# Autodesk Inventor assembly: encoder
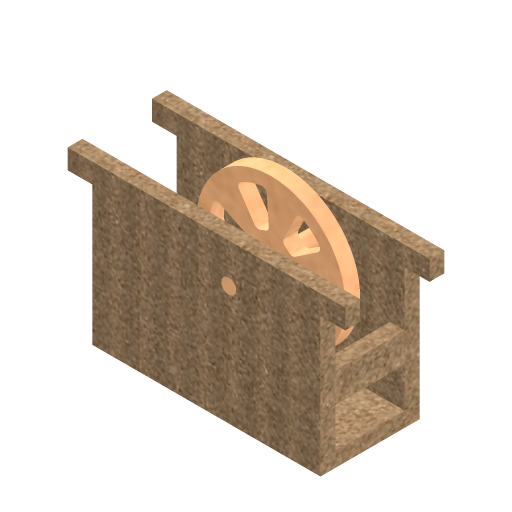
[picture p0: Inventor's stored thumbnail of the model, 512x512]
Saved by Autodesk Inventor 2024 (Build 280153000, 153)
## iProperties
Created: 2024-06-06
Document SubType Name: Assembly
Designer: USER
Author: 第26組
Title: encoder
## Documents named in this file (7)
- C:\Users\op04o\OneDrive\桌面\實務\final\圖檔\encoder\encoder.iam
- C:\Users\op04o\OneDrive\桌面\實務\final\圖檔\encoder\LM393.ipt
- C:\Users\op04o\OneDrive\桌面\實務\final\圖檔\encoder\wheel_6_hollow.ipt
- C:\Users\op04o\OneDrive\桌面\實務\final\圖檔\encoder\wheel_bar.ipt
- C:\Users\op04o\OneDrive\桌面\實務\final\圖檔\encoder\side_wall.ipt
- C:\Users\op04o\OneDrive\桌面\實務\final\圖檔\encoder\side_wall_short.ipt
- C:\Users\op04o\OneDrive\桌面\實務\final\圖檔\encoder\blocker.ipt
## Components (8 placed, 6 different names)
1. LM393:1 — Mate:1, Mate:3, Flush:1, Flush:2
2. wheel_6_hollow:1 — Mate:1, Mate:2
3. wheel_bar:1 — Mate:2, Mate:4, Flush:8
4. side_wall:1 — Mate:3, Flush:1, Flush:2, Mate:4, Flush:3, Mate:5, Flush:4, Angle:2, Mate:6, Flush:11, Flush:12
5. side_wall_short:1 — Flush:3, Mate:5, Flush:4, Flush:5, Flush:6, Flush:7
6. side_wall:2 — Flush:5, Flush:6, Flush:7, Flush:8, Mate:7
7. blocker:1 — Angle:1, Angle:2, Mate:6, Flush:9, Flush:10, Flush:11, Mate:7
8. blocker:2 — Angle:1, Flush:9, Flush:10, Flush:12
## Relationships (21: Flush 12, Mate 7, Angle 2)
- Mate:1 (1 mm): LM393:1 ↔ wheel_6_hollow:1
- Mate:2: wheel_6_hollow:1 ↔ wheel_bar:1
- Mate:3: LM393:1 ↔ side_wall:1
- Flush:1: LM393:1 ↔ side_wall:1
- Flush:2: LM393:1 ↔ side_wall:1
- Mate:4: wheel_bar:1 ↔ side_wall:1
- Flush:3: side_wall:1 ↔ side_wall_short:1
- Mate:5: side_wall:1 ↔ side_wall_short:1
- Flush:4: side_wall:1 ↔ side_wall_short:1
- Flush:5: side_wall_short:1 ↔ side_wall:2
- Flush:6: side_wall_short:1 ↔ side_wall:2
- Flush:7: side_wall_short:1 ↔ side_wall:2
- Flush:8: wheel_bar:1 ↔ side_wall:2
- Angle:1 (0 deg): blocker:1 ↔ blocker:2
- Angle:2 (0 deg): side_wall:1 ↔ blocker:1
- Mate:6: side_wall:1 ↔ blocker:1
- Flush:9: blocker:1 ↔ blocker:2
- Flush:10: blocker:1 ↔ blocker:2
- Flush:11: side_wall:1 ↔ blocker:1
- Flush:12: side_wall:1 ↔ blocker:2
- Mate:7: side_wall:2 ↔ blocker:1
